# Autodesk Inventor assembly: pen
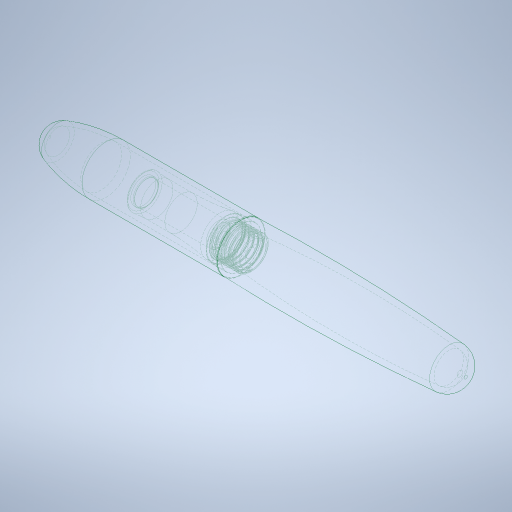
[picture p0: Inventor's stored thumbnail of the model, 512x512]
Saved by Autodesk Inventor 2024 (Build 280153000, 153)
## iProperties
Created: 2024-11-24
Part Number: pen
Document SubType Name: Assembly
Designer: Emil
Author: Emil
## Documents named in this file (4)
- C:\Users\Emil\OneDrive\Dokument\Projekt-Emil\Fountain_pen+Case+Pen_Holder\InventorCad\MyFountain_Pen\pen.iam
- C:\Users\Emil\OneDrive\Dokument\Projekt-Emil\Fountain_pen+Case+Pen_Holder\InventorCad\MyFountain_Pen\section\HongDian Nib Section.ipt
- C:\Users\Emil\OneDrive\Dokument\Projekt-Emil\Fountain_pen+Case+Pen_Holder\InventorCad\MyFountain_Pen\Body.ipt
- C:\Users\Emil\OneDrive\Dokument\Projekt-Emil\Fountain_pen+Case+Pen_Holder\InventorCad\MyFountain_Pen\Cap.ipt
## Components (3 placed, 3 different names)
1. HongDian Nib Section:1 — Rotational:1
2. Body:1 — Rotational:1, Rotational:2
3. Cap:1 — Rotational:2
## Relationships (2: RevoluteJoint 2)
- Rotational:1 [RevoluteJoint]: HongDian Nib Section:1 ↔ Body:1
- Rotational:2 [RevoluteJoint]: Body:1 ↔ Cap:1
